# Autodesk Inventor assembly: Case inferiore e batteria
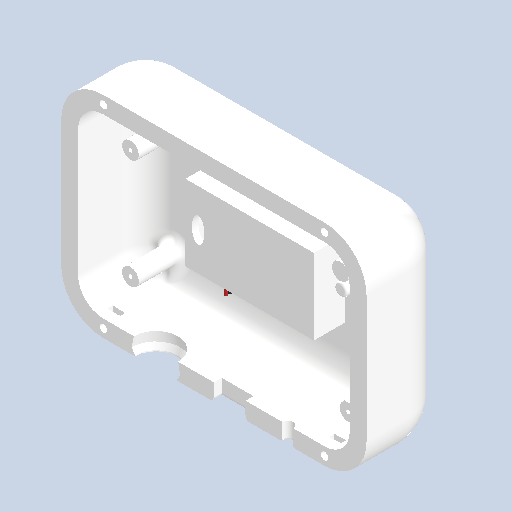
[picture p0: Inventor's stored thumbnail of the model, 512x512]
Saved by Autodesk Inventor 2023 (Build 270158000, 158)
## iProperties
Created: 2022-12-31
Part Number: Case inferiore e batteria
Document SubType Name: Assembly
Designer: Gabriele
Author: Gabriele
## Documents named in this file (3)
- C:\Users\Gabriele\Desktop\LAB\AY2223_I_Project-2\3D\Case\Case inferiore e batteria.iam
- C:\Users\Gabriele\Desktop\LAB\AY2223_I_Project-2\3D\Case\Case inferiore.ipt
- C:\Users\Gabriele\Desktop\LAB\AY2223_I_Project-2\3D\Case\Batteria e connettore.iam
## Components (2 placed, 2 different names)
1. Case inferiore:1 — Coincidente:1, Coincidente:2, Allineato:1
2. Batteria e connettore:1 [sub-assembly] — Coincidente:1, Coincidente:2, Allineato:1
## Relationships (3: Mate 2, Flush 1)
- Coincidente:1 [Mate] (9 mm): Case inferiore:1 ↔ Batteria e connettore:1
- Coincidente:2 [Mate] (2 mm): Case inferiore:1 ↔ Batteria e connettore:1
- Allineato:1 [Flush]: Case inferiore:1 ↔ Batteria e connettore:1
